# Autodesk Inventor assembly: Assembly6
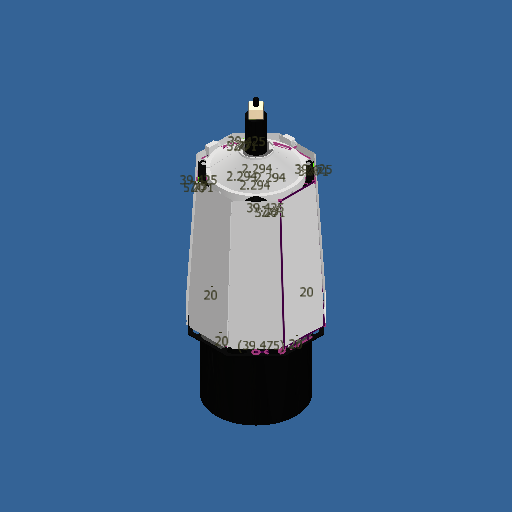
[picture p0: Inventor's stored thumbnail of the model, 512x512]
Saved by Autodesk Inventor 2026.2 (Build 302298000, 298)
## iProperties
Created: 2025-12-09
Part Number: Assembly6
Document SubType Name: Assembly
Designer: Thoma
Mass: 26734 g
Surface Area: 22861.5 cm^2
Volume: 10269 cm^3
Density: 2.60336 g/cm^3
Author: Thoma
## Documents named in this file (20)
- C:\Users\Thoma\OneDrive\Desktop\dir\telescope_cover\telescope\version_3\derive_rod_v6.iam
- C:\Users\Thoma\OneDrive\Desktop\dir\telescope_cover\telescope\version_3\Telescope_End.ipt
- C:\Users\Thoma\OneDrive\Desktop\dir\telescope_cover\telescope\version_3\Triangle.ipt
- C:\Users\Thoma\OneDrive\Desktop\dir\telescope_cover\telescope\version_3\Triangle_Bracket_Top.ipt
- C:\Users\Thoma\OneDrive\Desktop\dir\telescope_cover\telescope\version_3\Carbon_Fibre.ipt
- C:\Users\Thoma\OneDrive\Desktop\dir\telescope_cover\telescope\version_3\5mm Screw.ipt
- C:\Users\Thoma\OneDrive\Desktop\dir\telescope_cover\telescope\version_3\35mm_bolt.ipt
- C:\Users\Thoma\OneDrive\Desktop\dir\telescope_cover\telescope\version_3\Triangle_Bracket_Bottom_MIR.ipt
- C:\Users\Thoma\OneDrive\Desktop\dir\telescope_cover\telescope\version_3\Telescope_Base.ipt
- C:\Users\Thoma\OneDrive\Desktop\dir\telescope_cover\telescope\version_3\Full_shaft_Simplify_3.ipt
- C:\Users\Thoma\OneDrive\Desktop\dir\telescope_cover\main\version_2\Conic_Cover_Simplify_1.ipt
- C:\Users\Thoma\OneDrive\Desktop\dir\telescope_cover\telescope\version_3\30mm_bolt.ipt
- C:\Users\Thoma\OneDrive\Desktop\dir\telescope_cover\telescope\version_3\Baffle.ipt
- C:\Users\Thoma\OneDrive\Desktop\dir\telescope_cover\telescope\version_3\Bottom_End_Top.ipt
- C:\Users\Thoma\OneDrive\Desktop\dir\telescope_cover\main\version_2\Cover_Lower_v3.ipt
- C:\Users\Thoma\OneDrive\Desktop\dir\telescope_cover\main\version_2\Cover_Upper_v3.ipt
- C:\Users\Thoma\OneDrive\Desktop\dir\telescope_cover\telescope\version_3\4mm_0.5_Screw.ipt
- C:\Users\Thoma\OneDrive\Desktop\dir\telescope_cover\telescope\version_3\Base_Plate_v2.ipt
- C:\Users\Thoma\OneDrive\Desktop\dir\telescope_cover\servo\motor_basic.ipt
- C:\Users\Thoma\OneDrive\Desktop\dir\telescope_cover\telescope\version_3\rod_v4.iam
## Components (63 placed, 19 different names)
1. Cover_Lower_v3:1 — Flush:111, Flush:112, Flush:113
2. Cover_Upper_v3:1 — Flush:114, Flush:115, Flush:116, Mate:164, Mate:165, Tangent:19
3. Cover_Upper_v3:2 — Flush:117, Flush:118, Flush:119
4. Cover_Lower_v3:2 — Mate:145, Mate:146, Tangent:18, Mate:147, Mate:148, Mate:149, Mate:150, Mate:151, Mate:152
5. Base_Plate_v2:1 — Mate:141, Mate:142, Mate:143, Angle:64, Flush:135, Mate:155, Mate:156
6. motor_basic:1 — Angle:64, Flush:135, Mate:153, Mate:155, Mate:156, Mate:157
7. rod_v4:1 [sub-assembly] — Mate:145, Mate:146, Tangent:18, Angle:65, Angle:66, Angle:67, Mate:153, Mate:157
8. 4mm_0.5_Screw:1 — Mate:147, Mate:148, Angle:65
9. 4mm_0.5_Screw:2 — Mate:149, Mate:150, Angle:66
10. 4mm_0.5_Screw:3 — Mate:151, Mate:152, Angle:67
11. Base_Plate_v2:2 — Mate:158, Mate:159, Mate:160, Mate:163, Flush:136
12. motor_basic:2 — Mate:163, Flush:136
13. rod_v4:2 [sub-assembly] — Mate:164, Mate:165, Tangent:19
14. Baffle:1 — Mate:83
15. Carbon_Fibre:1 — Mate:7, Mate:11, Flush:1, Mate:12, Mate:13, Mate:14, Mate:15, Mate:32, Mate:33, Mate:62, Flush:2, Flush:3, Flush:4, Flush:5, Mate:83, Mate:92, Mate:93, Mate:95, Mate:96, Mate:97, Mate:98, Mate:99, Mate:100, Mate:123, Mate:124, Mate:125
16. Telescope_Base:1 — Mate:62, Angle:31, Mate:89, Mate:90, Angle:40, Mate:108, Mate:109, Angle:48, Mate:110, Mate:111, Angle:49, Mate:112, Mate:113, Angle:50
17. Telescope_End:1 — Mate:1, Mate:2, Angle:2, Mate:7, Mate:54, Mate:55, Angle:26, Angle:31, Mate:86, Mate:88, Mate:91, Angle:41, Mate:101, Angle:45, Angle:46, Mate:114, Mate:115, Angle:51, Mate:116, Mate:117, Angle:52, Mate:118, Mate:119, Angle:53, Mate:141, Mate:142, Mate:143, Mate:158, Mate:159, Mate:160
18. Triangle_Bracket_Top:5 — Mate:116, Mate:117, Angle:52, Mate:129, Flush:110, Angle:60
19. Triangle_Bracket_Top:4 — Mate:101, Angle:45, Angle:46, Mate:104, Mate:105, Mate:106, Flush:103, Angle:47, Flush:116
20. Triangle_Bracket_Top:3 — Mate:86, Mate:88, Mate:94, Angle:54, Angle:55, Mate:122, Flush:106, Angle:56
21. Triangle_Bracket_Top:1 — Mate:1, Mate:2, Angle:2, Mate:8, Mate:9, Angle:4, Mate:47, Angle:22, Mate:58, Flush:113, Flush:119
22. Triangle:1 — Mate:8, Mate:9, Angle:4, Mate:11, Flush:1, Angle:5, Angle:6, Mate:46, Mate:70, Mate:71, Flush:111, Flush:117
23. Triangle:5 — Angle:16, Mate:66, Mate:67, Mate:92, Mate:93, Mate:94, Flush:14, Angle:42, Mate:102, Mate:128, Flush:109, Angle:59, Mate:132, Flush:115
24. Triangle:6 — Mate:96, Mate:97, Mate:98, Flush:101, Angle:43, Flush:102, Angle:44, Mate:103, Mate:104, Mate:105, Mate:107, Flush:112, Flush:114
25. Triangle:7 — Mate:123, Mate:124, Mate:125, Mate:126, Flush:107, Angle:57, Mate:127, Flush:108, Angle:58, Mate:130, Mate:131, Flush:118
26. 35mm_bolt:6 — Mate:122, Flush:106, Angle:56
27. 35mm_bolt:7 — Mate:129, Flush:110, Angle:60
28. 35mm_bolt:4 — Mate:46, Mate:47, Angle:22
29. 35mm_bolt:5 — Mate:106, Flush:103, Angle:47
30. 5mm Screw:9 — Mate:100, Flush:102, Angle:44
31. 5mm Screw:8 — Mate:99, Flush:101, Angle:43
32. 5mm Screw:7 — Angle:16, Mate:32, Mate:33, Mate:95, Flush:14, Angle:42
33. 5mm Screw:10 — Mate:126, Flush:107, Angle:57
34. 5mm Screw:2 — Mate:14, Mate:15, Angle:6
35. 5mm Screw:1 — Mate:12, Mate:13, Angle:5
36. 5mm Screw:11 — Mate:127, Flush:108, Angle:58
37. 5mm Screw:12 — Mate:128, Flush:109, Angle:59
38. 30mm_bolt:7 — Mate:120, Flush:104, Angle:54
39. 30mm_bolt:1 — Mate:121, Flush:105, Angle:55
40. 30mm_bolt:8 — Mate:80, Flush:13, Angle:39
41. 30mm_bolt:6 — Mate:78, Flush:11, Angle:37
42. 30mm_bolt:3 — Mate:79, Flush:12, Angle:38
43. 30mm_bolt:2 — Mate:77, Flush:10, Angle:36
44. Triangle_Bracket_Bottom_MIR:4 — Mate:118, Mate:119, Angle:53, Tangent:15, Tangent:16
45. Triangle_Bracket_Bottom_MIR:3 — Mate:114, Mate:115, Angle:51, Mate:120, Flush:104, Mate:121, Flush:105, Tangent:14
46. Triangle_Bracket_Bottom_MIR:2 — Mate:55, Mate:58, Angle:26, Tangent:4, Mate:77, Flush:10, Angle:36, Mate:78, Flush:11, Angle:37, Tangent:17
47. Triangle_Bracket_Bottom_MIR:1 — Mate:54, Mate:79, Flush:12, Angle:38, Mate:80, Flush:13, Angle:39, Tangent:9, Mate:91, Angle:41, Tangent:13
48. Bottom_End_Top:4 — Mate:112, Mate:113, Angle:50
49. Bottom_End_Top:3 — Mate:110, Mate:111, Angle:49
50. Bottom_End_Top:2 — Mate:108, Mate:109, Angle:48
51. Bottom_End_Top:1 — Mate:89, Mate:90, Angle:40, Tangent:11
52. Full_shaft_Simplify_3:3
53. Full_shaft_Simplify_3:7 — Tangent:16
54. Full_shaft_Simplify_3:8 — Tangent:17
55. Full_shaft_Simplify_3:5 — Tangent:14
56. Full_shaft_Simplify_3:6 — Tangent:15
57. Full_shaft_Simplify_3:4 — Tangent:13
58. Full_shaft_Simplify_3:1 — Tangent:4, Tangent:11
59. Full_shaft_Simplify_3:2 — Tangent:9
60. Conic_Cover_Simplify_1:1 — Flush:2, Mate:66, Mate:131, Mate:132
61. Conic_Cover_Simplify_1:2 — Mate:67, Flush:3, Mate:102, Mate:103
62. Conic_Cover_Simplify_1:3 — Flush:4, Mate:70, Mate:107
63. Conic_Cover_Simplify_1:4 — Mate:71, Flush:5, Mate:130
## Relationships (172: Mate 94, Angle 37, Flush 31, Tangent 10)
- Mate:1: Telescope_End:1 ↔ Triangle_Bracket_Top:1
- Mate:2: Telescope_End:1 ↔ Triangle_Bracket_Top:1
- Angle:2 (0 deg): Telescope_End:1 ↔ Triangle_Bracket_Top:1
- Mate:7: Carbon_Fibre:1 ↔ Telescope_End:1
- Mate:8: Triangle_Bracket_Top:1 ↔ Triangle:1
- Mate:9: Triangle_Bracket_Top:1 ↔ Triangle:1
- Angle:4 (0 deg): Triangle_Bracket_Top:1 ↔ Triangle:1
- Mate:11: Carbon_Fibre:1 ↔ Triangle:1
- Flush:1: Carbon_Fibre:1 ↔ Triangle:1
- Mate:12: Carbon_Fibre:1 ↔ 5mm Screw:1
- Mate:13: Carbon_Fibre:1 ↔ 5mm Screw:1
- Angle:5 (0 deg): Triangle:1 ↔ 5mm Screw:1
- Mate:14: Carbon_Fibre:1 ↔ 5mm Screw:2
- Mate:15: Carbon_Fibre:1 ↔ 5mm Screw:2
- Angle:6 (0 deg): Triangle:1 ↔ 5mm Screw:2
- Angle:16 (0 deg): Triangle:5 ↔ 5mm Screw:7
- Mate:32: Carbon_Fibre:1 ↔ 5mm Screw:7
- Mate:33: Carbon_Fibre:1 ↔ 5mm Screw:7
- Mate:46: Triangle:1 ↔ 35mm_bolt:4
- Mate:47: Triangle_Bracket_Top:1 ↔ 35mm_bolt:4
- Angle:22 (0 deg): Triangle_Bracket_Top:1 ↔ 35mm_bolt:4
- Mate:54: Telescope_End:1 ↔ Triangle_Bracket_Bottom_MIR:1
- Mate:55: Telescope_End:1 ↔ Triangle_Bracket_Bottom_MIR:2
- Mate:58: Triangle_Bracket_Top:1 ↔ Triangle_Bracket_Bottom_MIR:2
- Angle:26 (0 deg): Telescope_End:1 ↔ Triangle_Bracket_Bottom_MIR:2
- Mate:62: Carbon_Fibre:1 ↔ Telescope_Base:1
- Angle:31 (0 deg): Telescope_Base:1 ↔ Telescope_End:1
- Tangent:4: Triangle_Bracket_Bottom_MIR:2 ↔ Full_shaft_Simplify_3:1
- Flush:2: Carbon_Fibre:1 ↔ Conic_Cover_Simplify_1:1
- Mate:66: Triangle:5 ↔ Conic_Cover_Simplify_1:1
- Mate:67: Triangle:5 ↔ Conic_Cover_Simplify_1:2
- Flush:3: Carbon_Fibre:1 ↔ Conic_Cover_Simplify_1:2
- Flush:4: Carbon_Fibre:1 ↔ Conic_Cover_Simplify_1:3
- Mate:70: Triangle:1 ↔ Conic_Cover_Simplify_1:3
- Mate:71: Triangle:1 ↔ Conic_Cover_Simplify_1:4
- Flush:5: Carbon_Fibre:1 ↔ Conic_Cover_Simplify_1:4
- Mate:77: 30mm_bolt:2 ↔ Triangle_Bracket_Bottom_MIR:2
- Flush:10: 30mm_bolt:2 ↔ Triangle_Bracket_Bottom_MIR:2
- Angle:36 (0 deg): 30mm_bolt:2 ↔ Triangle_Bracket_Bottom_MIR:2
- Mate:78: 30mm_bolt:6 ↔ Triangle_Bracket_Bottom_MIR:2
- Flush:11: 30mm_bolt:6 ↔ Triangle_Bracket_Bottom_MIR:2
- Angle:37 (0 deg): 30mm_bolt:6 ↔ Triangle_Bracket_Bottom_MIR:2
- Mate:79: 30mm_bolt:3 ↔ Triangle_Bracket_Bottom_MIR:1
- Flush:12: 30mm_bolt:3 ↔ Triangle_Bracket_Bottom_MIR:1
- Angle:38 (0 deg): 30mm_bolt:3 ↔ Triangle_Bracket_Bottom_MIR:1
- Mate:80: 30mm_bolt:8 ↔ Triangle_Bracket_Bottom_MIR:1
- Flush:13: 30mm_bolt:8 ↔ Triangle_Bracket_Bottom_MIR:1
- Angle:39 (0 deg): 30mm_bolt:8 ↔ Triangle_Bracket_Bottom_MIR:1
- Mate:83: Baffle:1 ↔ Carbon_Fibre:1
- Tangent:9: Triangle_Bracket_Bottom_MIR:1 ↔ Full_shaft_Simplify_3:2
- Mate:86: Telescope_End:1 ↔ Triangle_Bracket_Top:3
- Mate:88: Telescope_End:1 ↔ Triangle_Bracket_Top:3
- Mate:89: Telescope_Base:1 ↔ Bottom_End_Top:1
- Mate:90: Telescope_Base:1 ↔ Bottom_End_Top:1
- Angle:40 (0 deg): Telescope_Base:1 ↔ Bottom_End_Top:1
- Tangent:11: Bottom_End_Top:1 ↔ Full_shaft_Simplify_3:1
- Mate:91: Telescope_End:1 ↔ Triangle_Bracket_Bottom_MIR:1
- Angle:41 (0 deg): Telescope_End:1 ↔ Triangle_Bracket_Bottom_MIR:1
- Mate:92: Carbon_Fibre:1 ↔ Triangle:5
- Mate:93: Carbon_Fibre:1 ↔ Triangle:5
- Mate:94: Triangle_Bracket_Top:3 ↔ Triangle:5
- Mate:95: Carbon_Fibre:1 ↔ 5mm Screw:7
- Flush:14: Triangle:5 ↔ 5mm Screw:7
- Angle:42 (0 deg): Triangle:5 ↔ 5mm Screw:7
- Mate:96: Carbon_Fibre:1 ↔ Triangle:6
- Mate:97: Carbon_Fibre:1 ↔ Triangle:6
- Mate:98: Carbon_Fibre:1 ↔ Triangle:6
- Mate:99: Carbon_Fibre:1 ↔ 5mm Screw:8
- Flush:101: Triangle:6 ↔ 5mm Screw:8
- Angle:43 (0 deg): Triangle:6 ↔ 5mm Screw:8
- Mate:100: Carbon_Fibre:1 ↔ 5mm Screw:9
- Flush:102: Triangle:6 ↔ 5mm Screw:9
- Angle:44 (0 deg): Triangle:6 ↔ 5mm Screw:9
- Mate:101: Telescope_End:1 ↔ Triangle_Bracket_Top:4
- Angle:45 (0 deg): Telescope_End:1 ↔ Triangle_Bracket_Top:4
- Mate:102: Triangle:5 ↔ Conic_Cover_Simplify_1:2
- Mate:103: Triangle:6 ↔ Conic_Cover_Simplify_1:2
- Angle:46 (0 deg): Telescope_End:1 ↔ Triangle_Bracket_Top:4
- Mate:104: Triangle_Bracket_Top:4 ↔ Triangle:6
- Mate:105: Triangle_Bracket_Top:4 ↔ Triangle:6
- Mate:106: Triangle_Bracket_Top:4 ↔ 35mm_bolt:5
- Flush:103: Triangle_Bracket_Top:4 ↔ 35mm_bolt:5
- Angle:47 (0 deg): Triangle_Bracket_Top:4 ↔ 35mm_bolt:5
- Mate:107: Triangle:6 ↔ Conic_Cover_Simplify_1:3
- Mate:108: Telescope_Base:1 ↔ Bottom_End_Top:2
- Mate:109: Telescope_Base:1 ↔ Bottom_End_Top:2
- Angle:48 (0 deg): Telescope_Base:1 ↔ Bottom_End_Top:2
- Mate:110: Telescope_Base:1 ↔ Bottom_End_Top:3
- Mate:111: Telescope_Base:1 ↔ Bottom_End_Top:3
- Angle:49 (0 deg): Telescope_Base:1 ↔ Bottom_End_Top:3
- Mate:112: Telescope_Base:1 ↔ Bottom_End_Top:4
- Mate:113: Telescope_Base:1 ↔ Bottom_End_Top:4
- Angle:50 (0 deg): Telescope_Base:1 ↔ Bottom_End_Top:4
- Mate:114: Telescope_End:1 ↔ Triangle_Bracket_Bottom_MIR:3
- Mate:115: Telescope_End:1 ↔ Triangle_Bracket_Bottom_MIR:3
- Angle:51 (0 deg): Telescope_End:1 ↔ Triangle_Bracket_Bottom_MIR:3
- Tangent:13: Triangle_Bracket_Bottom_MIR:1 ↔ Full_shaft_Simplify_3:4
- Mate:116: Telescope_End:1 ↔ Triangle_Bracket_Top:5
- Mate:117: Telescope_End:1 ↔ Triangle_Bracket_Top:5
- Angle:52 (0 deg): Telescope_End:1 ↔ Triangle_Bracket_Top:5
- Mate:118: Telescope_End:1 ↔ Triangle_Bracket_Bottom_MIR:4
- Mate:119: Telescope_End:1 ↔ Triangle_Bracket_Bottom_MIR:4
- Angle:53 (0 deg): Telescope_End:1 ↔ Triangle_Bracket_Bottom_MIR:4
- Mate:120: 30mm_bolt:7 ↔ Triangle_Bracket_Bottom_MIR:3
- Flush:104: 30mm_bolt:7 ↔ Triangle_Bracket_Bottom_MIR:3
- Angle:54 (0 deg): Triangle_Bracket_Top:3 ↔ 30mm_bolt:7
- Mate:121: 30mm_bolt:1 ↔ Triangle_Bracket_Bottom_MIR:3
- Flush:105: 30mm_bolt:1 ↔ Triangle_Bracket_Bottom_MIR:3
- Angle:55 (0 deg): Triangle_Bracket_Top:3 ↔ 30mm_bolt:1
- Mate:122: Triangle_Bracket_Top:3 ↔ 35mm_bolt:6
- Flush:106: Triangle_Bracket_Top:3 ↔ 35mm_bolt:6
- Angle:56 (0 deg): Triangle_Bracket_Top:3 ↔ 35mm_bolt:6
- Mate:123: Carbon_Fibre:1 ↔ Triangle:7
- Mate:124: Carbon_Fibre:1 ↔ Triangle:7
- Mate:125: Carbon_Fibre:1 ↔ Triangle:7
- Mate:126: Triangle:7 ↔ 5mm Screw:10
- Flush:107: Triangle:7 ↔ 5mm Screw:10
- Angle:57 (0 deg): Triangle:7 ↔ 5mm Screw:10
- Mate:127: Triangle:7 ↔ 5mm Screw:11
- Flush:108: Triangle:7 ↔ 5mm Screw:11
- Angle:58 (0 deg): Triangle:7 ↔ 5mm Screw:11
- Mate:128: Triangle:5 ↔ 5mm Screw:12
- Flush:109: Triangle:5 ↔ 5mm Screw:12
- Angle:59 (0 deg): Triangle:5 ↔ 5mm Screw:12
- Mate:129: Triangle_Bracket_Top:5 ↔ 35mm_bolt:7
- Flush:110: Triangle_Bracket_Top:5 ↔ 35mm_bolt:7
- Angle:60 (0 deg): Triangle_Bracket_Top:5 ↔ 35mm_bolt:7
- Tangent:14: Triangle_Bracket_Bottom_MIR:3 ↔ Full_shaft_Simplify_3:5
- Tangent:15: Triangle_Bracket_Bottom_MIR:4 ↔ Full_shaft_Simplify_3:6
- Tangent:16: Triangle_Bracket_Bottom_MIR:4 ↔ Full_shaft_Simplify_3:7
- Tangent:17: Triangle_Bracket_Bottom_MIR:2 ↔ Full_shaft_Simplify_3:8
- Mate:130: Triangle:7 ↔ Conic_Cover_Simplify_1:4
- Mate:131: Triangle:7 ↔ Conic_Cover_Simplify_1:1
- Mate:132: Triangle:5 ↔ Conic_Cover_Simplify_1:1
- Flush:111: Cover_Lower_v3:1 ↔ Triangle:1
- Flush:112: Cover_Lower_v3:1 ↔ Triangle:6
- Flush:113 (2 mm): Cover_Lower_v3:1 ↔ Triangle_Bracket_Top:1
- Flush:114: Cover_Upper_v3:1 ↔ Triangle:6
- Flush:115: Cover_Upper_v3:1 ↔ Triangle:5
- Flush:116 (2 mm): Cover_Upper_v3:1 ↔ Triangle_Bracket_Top:4
- Flush:117: Cover_Upper_v3:2 ↔ Triangle:1
- Flush:118: Cover_Upper_v3:2 ↔ Triangle:7
- Flush:119 (2 mm): Cover_Upper_v3:2 ↔ Triangle_Bracket_Top:1
- Mate:141: Base_Plate_v2:1 ↔ Telescope_End:1
- Mate:142: Base_Plate_v2:1 ↔ Telescope_End:1
- Mate:143: Base_Plate_v2:1 ↔ Telescope_End:1
- Angle:64 (0 deg): Base_Plate_v2:1 ↔ motor_basic:1
- Flush:135: Base_Plate_v2:1 ↔ motor_basic:1
- Mate:145: Cover_Lower_v3:2 ↔ rod_v4:1
- Mate:146: Cover_Lower_v3:2 ↔ rod_v4:1
- Tangent:18: Cover_Lower_v3:2 ↔ rod_v4:1
- Mate:147: Cover_Lower_v3:2 ↔ 4mm_0.5_Screw:1
- Mate:148: Cover_Lower_v3:2 ↔ 4mm_0.5_Screw:1
- Angle:65 (10 deg): rod_v4:1 ↔ 4mm_0.5_Screw:1
- Mate:149: Cover_Lower_v3:2 ↔ 4mm_0.5_Screw:2
- Mate:150: Cover_Lower_v3:2 ↔ 4mm_0.5_Screw:2
- Mate:151: Cover_Lower_v3:2 ↔ 4mm_0.5_Screw:3
- Mate:152: Cover_Lower_v3:2 ↔ 4mm_0.5_Screw:3
- Angle:66 (0 deg): rod_v4:1 ↔ 4mm_0.5_Screw:2
- Angle:67 (0 deg): rod_v4:1 ↔ 4mm_0.5_Screw:3
- Mate:153: motor_basic:1 ↔ rod_v4:1
- Mate:155: Base_Plate_v2:1 ↔ motor_basic:1
- Mate:156 (-53 mm): Base_Plate_v2:1 ↔ motor_basic:1
- Mate:157 (2 mm): motor_basic:1 ↔ rod_v4:1
- Mate:158: Base_Plate_v2:2 ↔ Telescope_End:1
- Mate:159: Base_Plate_v2:2 ↔ Telescope_End:1
- Mate:160: Base_Plate_v2:2 ↔ Telescope_End:1
- Mate:163: Base_Plate_v2:2 ↔ motor_basic:2
- Flush:136: Base_Plate_v2:2 ↔ motor_basic:2
- Mate:164: Cover_Upper_v3:1 ↔ rod_v4:2
- Mate:165: Cover_Upper_v3:1 ↔ rod_v4:2
- Tangent:19 (-1 mm): Cover_Upper_v3:1 ↔ rod_v4:2
